# Autodesk Inventor assembly: Steering Electrical Assembly
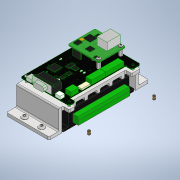
[picture p0: Inventor's stored thumbnail of the model, 180x180]
Saved by Autodesk Inventor 2020 (Build 240168000, 168)
## iProperties
Created: 2019-11-19
Part Number: Steering Electrical Assembly
Document SubType Name: Assembly
Designer: kylew
Author: kylew
## Documents named in this file (12)
- C:\Users\kylew\Documents\GitHub\roboracing-electrical\new-cari\Steering\Mounting CAD\Steering Electrical Assembly.iam
- C:\Users\kylew\Documents\GitHub\roboracing-electrical\new-cari\Steering\Mounting CAD\Aluminum_Heatsink_Base.ipt
- C:\Users\kylew\Documents\GitHub\roboracing-electrical\new-cari\Steering\Mounting CAD\CL57T_Stepper_Driver.ipt
- C:\Users\kylew\Documents\GitHub\roboracing-electrical\new-cari\Steering\Mounting CAD\Plastic_Bracket.ipt
- C:\Users\kylew\Documents\GitHub\roboracing-electrical\new-cari\Steering\Mounting CAD\ethernet_poe.brd.ipt
- C:\Users\kylew\Documents\GitHub\roboracing-electrical\new-cari\Steering\Mounting CAD\Steering.brd.ipt
- C:\Users\kylew\Documents\GitHub\roboracing-electrical\new-cari\Steering\Mounting CAD\M3_5mm_Insert.ipt
- C:\Users\kylew\Documents\GitHub\roboracing-electrical\new-cari\Steering\Mounting CAD\93657A207_NYLON UNTHREADED SPACER.ipt
- C:\Users\kylew\Documents\GitHub\roboracing-electrical\new-cari\Steering\Mounting CAD\92000A120_18-8 SS METRIC PAN HEAD PHIL MACHINE SCREW.ipt
- C:\Users\kylew\Documents\GitHub\roboracing-electrical\new-cari\Steering\Mounting CAD\92095A208_18-8 SS BUTTON-HEAD SOCKET CAP SCREW.ipt
- C:\Users\kylew\Documents\GitHub\roboracing-electrical\new-cari\Steering\Mounting CAD\92000A114_18-8 SS METRIC PAN HEAD PHIL MACHINE SCREW.ipt
- C:\Users\kylew\Documents\GitHub\roboracing-electrical\new-cari\Steering\Mounting CAD\95947A509_ALUM FEM THRDED HEX STANDOFF.ipt
## Components (33 placed, 11 different names)
1. Aluminum_Heatsink_Base:1 — Mate:1, Flush:1, Flush:2, Mate:2, Mate:3, Mate:33
2. CL57T_Stepper_Driver:1 — Mate:1, Flush:1, Flush:2, Mate:34, Mate:36
3. Plastic_Bracket:1 — Mate:2, Mate:3, Mate:6, Mate:9, Mate:10, Mate:11, Flush:3, Mate:12, Flush:4, Mate:13, Flush:5, Mate:14, Flush:6, Mate:15, Mate:18, Mate:19, Mate:20, Mate:32, Mate:35, Mate:36
4. ethernet_poe.brd:1 — Mate:5, Mate:7, Mate:8, Mate:39, Mate:40
5. Steering.brd:1 — Mate:5, Mate:6, Mate:7, Mate:8, Mate:9, Mate:10, Mate:23, Mate:24, Mate:25, Mate:26, Mate:27, Mate:28, Mate:29, Mate:30, Mate:41, Mate:42
6. M3_5mm_Insert:1 — Mate:12, Flush:4, Mate:17
7. M3_5mm_Insert:2 — Mate:11, Flush:3, Mate:16
8. M3_5mm_Insert:3 — Mate:14, Flush:6, Mate:22
9. M3_5mm_Insert:4 — Mate:13, Flush:5, Mate:21
10. 93657A207_NYLON UNTHREADED SPACER:1 — Mate:17, Mate:18
11. 93657A207_NYLON UNTHREADED SPACER:2 — Mate:19, Mate:21
12. 93657A207_NYLON UNTHREADED SPACER:3 — Mate:20, Mate:22
13. 93657A207_NYLON UNTHREADED SPACER:4 — Mate:15, Mate:16
14. 92000A120_18-8 SS METRIC PAN HEAD PHIL MACHINE SCREW:1 — Mate:25, Mate:26
15. 92000A120_18-8 SS METRIC PAN HEAD PHIL MACHINE SCREW:2 — Mate:23, Mate:24
16. 92000A120_18-8 SS METRIC PAN HEAD PHIL MACHINE SCREW:3 — Mate:27, Mate:28
17. 92000A120_18-8 SS METRIC PAN HEAD PHIL MACHINE SCREW:4 — Mate:29, Mate:30
18. M3_5mm_Insert:5
19. M3_5mm_Insert:6
20. 92095A208_18-8 SS BUTTON-HEAD SOCKET CAP SCREW:5 — Mate:33, Mate:34
21. 92095A208_18-8 SS BUTTON-HEAD SOCKET CAP SCREW:9
22. 92095A208_18-8 SS BUTTON-HEAD SOCKET CAP SCREW:10
23. 92095A208_18-8 SS BUTTON-HEAD SOCKET CAP SCREW:11
24. 92095A208_18-8 SS BUTTON-HEAD SOCKET CAP SCREW:8 — Mate:32, Mate:35
25. 92095A208_18-8 SS BUTTON-HEAD SOCKET CAP SCREW:12
26. 92095A208_18-8 SS BUTTON-HEAD SOCKET CAP SCREW:13
27. 92095A208_18-8 SS BUTTON-HEAD SOCKET CAP SCREW:14
28. 92000A114_18-8 SS METRIC PAN HEAD PHIL MACHINE SCREW:1 — Mate:39, Mate:40, Mate:43
29. 95947A509_ALUM FEM THRDED HEX STANDOFF:1 — Mate:42, Mate:43, Mate:44
30. 92000A114_18-8 SS METRIC PAN HEAD PHIL MACHINE SCREW:2 — Mate:41, Mate:44
31. 92000A114_18-8 SS METRIC PAN HEAD PHIL MACHINE SCREW:3
32. 95947A509_ALUM FEM THRDED HEX STANDOFF:2
33. 92000A114_18-8 SS METRIC PAN HEAD PHIL MACHINE SCREW:4
## Component patterns: (4 elements, first: 92095A208_18-8 SS BUTTON-HEAD SOCKET CAP SCREW:5), (4 elements, first: 92095A208_18-8 SS BUTTON-HEAD SOCKET CAP SCREW:8), (2 elements, first: 92000A114_18-8 SS METRIC PAN HEAD PHIL MACHINE SCREW:1 + 95947A509_ALUM FEM THRDED HEX STANDOFF:1 + 92000A114_18-8 SS METRIC PAN HEAD PHIL MACHINE SCREW:2)
## Relationships (46: Mate 40, Flush 6)
- Mate:1: Aluminum_Heatsink_Base:1 ↔ CL57T_Stepper_Driver:1
- Flush:1 (42 mm): Aluminum_Heatsink_Base:1 ↔ CL57T_Stepper_Driver:1
- Flush:2 (15.4 mm): Aluminum_Heatsink_Base:1 ↔ CL57T_Stepper_Driver:1
- Mate:2: Aluminum_Heatsink_Base:1 ↔ Plastic_Bracket:1
- Mate:3 (15.4 mm): Aluminum_Heatsink_Base:1 ↔ Plastic_Bracket:1
- Mate:5 (11 mm): ethernet_poe.brd:1 ↔ Steering.brd:1
- Mate:6 (5 mm): Plastic_Bracket:1 ↔ Steering.brd:1
- Mate:7: ethernet_poe.brd:1 ↔ Steering.brd:1
- Mate:8: ethernet_poe.brd:1 ↔ Steering.brd:1
- Mate:9: Plastic_Bracket:1 ↔ Steering.brd:1
- Mate:10: Plastic_Bracket:1 ↔ Steering.brd:1
- Mate:11: Plastic_Bracket:1 ↔ M3_5mm_Insert:2
- Flush:3: Plastic_Bracket:1 ↔ M3_5mm_Insert:2
- Mate:12: Plastic_Bracket:1 ↔ M3_5mm_Insert:1
- Flush:4: Plastic_Bracket:1 ↔ M3_5mm_Insert:1
- Mate:13: Plastic_Bracket:1 ↔ M3_5mm_Insert:4
- Flush:5: Plastic_Bracket:1 ↔ M3_5mm_Insert:4
- Mate:14: Plastic_Bracket:1 ↔ M3_5mm_Insert:3
- Flush:6: Plastic_Bracket:1 ↔ M3_5mm_Insert:3
- Mate:15: Plastic_Bracket:1 ↔ 93657A207_NYLON UNTHREADED SPACER:4
- Mate:16: M3_5mm_Insert:2 ↔ 93657A207_NYLON UNTHREADED SPACER:4
- Mate:17: M3_5mm_Insert:1 ↔ 93657A207_NYLON UNTHREADED SPACER:1
- Mate:18: Plastic_Bracket:1 ↔ 93657A207_NYLON UNTHREADED SPACER:1
- Mate:19: Plastic_Bracket:1 ↔ 93657A207_NYLON UNTHREADED SPACER:2
- Mate:20: Plastic_Bracket:1 ↔ 93657A207_NYLON UNTHREADED SPACER:3
- Mate:21: M3_5mm_Insert:4 ↔ 93657A207_NYLON UNTHREADED SPACER:2
- Mate:22: M3_5mm_Insert:3 ↔ 93657A207_NYLON UNTHREADED SPACER:3
- Mate:23: Steering.brd:1 ↔ 92000A120_18-8 SS METRIC PAN HEAD PHIL MACHINE SCREW:2
- Mate:24: Steering.brd:1 ↔ 92000A120_18-8 SS METRIC PAN HEAD PHIL MACHINE SCREW:2
- Mate:25: Steering.brd:1 ↔ 92000A120_18-8 SS METRIC PAN HEAD PHIL MACHINE SCREW:1
- Mate:26: Steering.brd:1 ↔ 92000A120_18-8 SS METRIC PAN HEAD PHIL MACHINE SCREW:1
- Mate:27: Steering.brd:1 ↔ 92000A120_18-8 SS METRIC PAN HEAD PHIL MACHINE SCREW:3
- Mate:28: Steering.brd:1 ↔ 92000A120_18-8 SS METRIC PAN HEAD PHIL MACHINE SCREW:3
- Mate:29: Steering.brd:1 ↔ 92000A120_18-8 SS METRIC PAN HEAD PHIL MACHINE SCREW:4
- Mate:30: Steering.brd:1 ↔ 92000A120_18-8 SS METRIC PAN HEAD PHIL MACHINE SCREW:4
- Mate:32: Plastic_Bracket:1 ↔ 92095A208_18-8 SS BUTTON-HEAD SOCKET CAP SCREW:8
- Mate:33: Aluminum_Heatsink_Base:1 ↔ 92095A208_18-8 SS BUTTON-HEAD SOCKET CAP SCREW:5
- Mate:34: CL57T_Stepper_Driver:1 ↔ 92095A208_18-8 SS BUTTON-HEAD SOCKET CAP SCREW:5
- Mate:35: Plastic_Bracket:1 ↔ 92095A208_18-8 SS BUTTON-HEAD SOCKET CAP SCREW:8
- Mate:36 (2 mm): CL57T_Stepper_Driver:1 ↔ Plastic_Bracket:1
- Mate:39: ethernet_poe.brd:1 ↔ 92000A114_18-8 SS METRIC PAN HEAD PHIL MACHINE SCREW:1
- Mate:40: ethernet_poe.brd:1 ↔ 92000A114_18-8 SS METRIC PAN HEAD PHIL MACHINE SCREW:1
- Mate:41: Steering.brd:1 ↔ 92000A114_18-8 SS METRIC PAN HEAD PHIL MACHINE SCREW:2
- Mate:42: Steering.brd:1 ↔ 95947A509_ALUM FEM THRDED HEX STANDOFF:1
- Mate:43: 92000A114_18-8 SS METRIC PAN HEAD PHIL MACHINE SCREW:1 ↔ 95947A509_ALUM FEM THRDED HEX STANDOFF:1
- Mate:44: 95947A509_ALUM FEM THRDED HEX STANDOFF:1 ↔ 92000A114_18-8 SS METRIC PAN HEAD PHIL MACHINE SCREW:2
